# Autodesk Inventor assembly: 200-10-ROCKER-BEARING-PROFILE-CONN-ASM-02
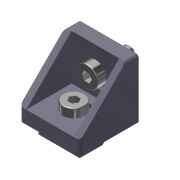
[picture p0: Inventor's stored thumbnail of the model, 180x180]
Saved by Autodesk Inventor 2018.2 (Build 222227000, 227)
## iProperties
Manager: feesmrt
Company: FRANCOR
Created: 2017-12-16
Part Number: 200-10-ROCKER-BEARING-PROFILE-CONN-ASM-02
Material: Generisch
Document SubType Name: Assembly
Designer: feesmrt
Project: Rescue Robot
Cost Center: -
Description: Rocker Bearing Profile Connector ASM
Engineer: feesmrt
Authority: feesmrt
Stock Number: 200-10-ROCKER-BEARING-PROFILE-CONN-ASM-01
Author: feesmrt
Title: Rocker Bearing Profile Connector ASM
Subject: Rescue Robot
Revision Number: 1
## Documents named in this file (5)
- D:\Programmierung\FRANC0R\CAD\02-Rocker-Bogie-Robot\200-ROCKER-BOGIE\200-10-ROCKER-BEARING\200-10-ROCKER-BEARING-PROFILE-CONN-ASM-02.iam
- D:\Programmierung\FRANC0R\CAD\02-Rocker-Bogie-Robot\900-COMPONENTS\900-50-PROFILES\900-50-PROFILES-ANGLE-CONN-30x30.ipt
- D:\Programmierung\FRANC0R\CAD\02-Rocker-Bogie-Robot\900-COMPONENTS\900-40-SCREWS\900-40-SCREWS-DIN7984_M6x16.ipt
- D:\Programmierung\FRANC0R\CAD\02-Rocker-Bogie-Robot\900-COMPONENTS\900-40-SCREWS\900-40-SCREWS-DIN7984_M6x12.ipt
- D:\Programmierung\FRANC0R\CAD\02-Rocker-Bogie-Robot\900-COMPONENTS\900-50-PROFILES\900-50-PROFILES-CONN-N8xM6.ipt
## Components (4 placed, 4 different names)
1. 900-50-PROFILES-ANGLE-CONN-30x30:1 — Passend:1, Passend:2, Fluchtend:1, Passend:3, Passend:4, Passend:5, Passend:7, Winkel:1
2. 900-40-SCREWS-DIN7984_M6x16:1 — Passend:1, Passend:2, Fluchtend:1
3. 900-40-SCREWS-DIN7984_M6x12:1 — Passend:3, Passend:4, Passend:5, Passend:6
4. 900-50-PROFILES-CONN-N8xM6:1 — Passend:6, Passend:7, Winkel:1
## Relationships (9: Mate 7, Flush 1, Angle 1)
- Passend:1 [Mate]: 900-50-PROFILES-ANGLE-CONN-30x30:1 ↔ 900-40-SCREWS-DIN7984_M6x16:1
- Passend:2 [Mate]: 900-50-PROFILES-ANGLE-CONN-30x30:1 ↔ 900-40-SCREWS-DIN7984_M6x16:1
- Fluchtend:1 [Flush] (16 mm): 900-50-PROFILES-ANGLE-CONN-30x30:1 ↔ 900-40-SCREWS-DIN7984_M6x16:1
- Passend:3 [Mate]: 900-50-PROFILES-ANGLE-CONN-30x30:1 ↔ 900-40-SCREWS-DIN7984_M6x12:1
- Passend:4 [Mate]: 900-50-PROFILES-ANGLE-CONN-30x30:1 ↔ 900-40-SCREWS-DIN7984_M6x12:1
- Passend:5 [Mate] (-16 mm): 900-50-PROFILES-ANGLE-CONN-30x30:1 ↔ 900-40-SCREWS-DIN7984_M6x12:1
- Passend:6 [Mate]: 900-40-SCREWS-DIN7984_M6x12:1 ↔ 900-50-PROFILES-CONN-N8xM6:1
- Passend:7 [Mate] (2.8 mm): 900-50-PROFILES-ANGLE-CONN-30x30:1 ↔ 900-50-PROFILES-CONN-N8xM6:1
- Winkel:1 [Angle] (0 deg): 900-50-PROFILES-ANGLE-CONN-30x30:1 ↔ 900-50-PROFILES-CONN-N8xM6:1
